# Autodesk Inventor assembly: LiftGearBeltConstruction
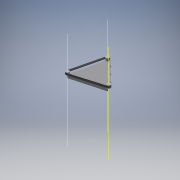
[picture p0: Inventor's stored thumbnail of the model, 180x180]
Saved by Autodesk Inventor 2018.3 (Build 223284000, 284)
## iProperties
Created: 2018-09-15
Part Number: LiftGearBeltConstruction
Material: Generisch
Document SubType Name: Assembly
Designer: JochenAlt
Author: JochenAlt
## Documents named in this file (3)
- D:\Projects\Ondine\CAD\Spindle\LiftGearBeltConstruction.iam
- D:\Projects\Ondine\CAD\Spindle\LiftGearBeltConstruction\Konstruktions-Assistent\Übertragung des Zahnriemens1.iam
- D:\Projects\Ondine\CAD\Spindle\LiftGearBeltConstruction\Konstruktions-Assistent\Bauteil7.ipt
## Components (2 placed, 2 different names)
1. Bauteil7:1 — Passend:1, Passend:2
2. Übertragung des Zahnriemens:1 [sub-assembly] — Passend:1, Passend:2
## Relationships (2: Mate 2)
- Passend:1 [Mate]: Bauteil7:1 ↔ Übertragung des Zahnriemens:1
- Passend:2 [Mate]: Bauteil7:1 ↔ Übertragung des Zahnriemens:1
